# Autodesk Inventor assembly: DriveSide_6inchWheels
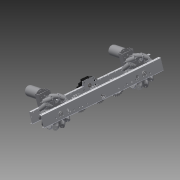
[picture p0: Inventor's stored thumbnail of the model, 180x180]
Saved by Autodesk Inventor 2015 (Build 190159000, 159)
## iProperties
Created: 2016-01-10
Part Number: DriveSide_6inchWheels
Document SubType Name: Assembly
Designer: Applefamily
Author: Applefamily
## Documents named in this file (10)
- C:\Users\Applegate\Desktop\Chassy_Wheeled\Assembly\DriveSide_6inchWheels.iam
- C:\Users\Applegate\Desktop\Chassy_Wheeled\Assembly\Imported Components\am-2951 AM14U2 Outside Sheet.ipt\am-2951 AM14U2 Outside Sheet.ipt.ipt
- C:\Users\Applegate\Desktop\Chassy_Wheeled\Assembly\GearBox and Mec.iam
- C:\Users\Applegate\Desktop\Chassy_Wheeled\Assembly\Imported Components\FR8ZZ Hex Bearing.ipt\FR8ZZ Hex Bearing.ipt.ipt
- C:\Users\Applegate\Desktop\Chassy_Wheeled\Assembly\Imported Components\am-2952 AM14U2 Inside Sheet.ipt\am-2952 AM14U2 Inside Sheet.ipt.ipt
- C:\Users\Applegate\Downloads\Imported Components\4 in HiGrip Wheel\4 in HiGrip Wheel.iam
- C:\Users\Applegate\Downloads\Imported Components\AM14U3+Long+REV1-1\am-2598_107 2016 KOP Toughbox Mini.iam
- am-2951 AM14U2 Outside Sheet.ipt
- FR8ZZ Hex Bearing.ipt
- am-2952 AM14U2 Inside Sheet.ipt
## Components (10 placed, 6 different names)
1. am-2951 AM14U2 Outside Sheet.ipt:1 — Cylindrical:1, Cylindrical:2, Mate:1, Mate:2, Cylindrical:7
2. GearBox and Mec:1 [sub-assembly] — Cylindrical:4, Cylindrical:6, Flush:1, Mate:3
3. FR8ZZ Hex Bearing.ipt:1 — Cylindrical:1, Mate:1, Cylindrical:6
4. FR8ZZ Hex Bearing.ipt:2 — Cylindrical:2, Mate:2, Cylindrical:3
5. GearBox and Mec:2 [sub-assembly] — Cylindrical:3, Cylindrical:5, Flush:1, Mate:4
6. am-2952 AM14U2 Inside Sheet.ipt:1 — Cylindrical:4, Cylindrical:5, Mate:3, Mate:4, Rotational:1
7. 4 in HiGrip Wheel:1 [sub-assembly] — Cylindrical:7, Flush:2, Flush:3
8. 4 in HiGrip Wheel:2 [sub-assembly] — Flush:2
9. 4 in HiGrip Wheel:3 [sub-assembly] — Flush:3
10. am-2598_107 2016 KOP Toughbox Mini:1 [sub-assembly] — Rotational:1
## Relationships (15: CylindricalJoint 7, Mate 4, Flush 3, RevoluteJoint 1)
- Cylindrical:1: am-2951 AM14U2 Outside Sheet.ipt:1 ↔ FR8ZZ Hex Bearing.ipt:1
- Cylindrical:2: am-2951 AM14U2 Outside Sheet.ipt:1 ↔ FR8ZZ Hex Bearing.ipt:2
- Mate:1: am-2951 AM14U2 Outside Sheet.ipt:1 ↔ FR8ZZ Hex Bearing.ipt:1
- Mate:2: am-2951 AM14U2 Outside Sheet.ipt:1 ↔ FR8ZZ Hex Bearing.ipt:2
- Cylindrical:3: FR8ZZ Hex Bearing.ipt:2 ↔ GearBox and Mec:2
- Cylindrical:4: GearBox and Mec:1 ↔ am-2952 AM14U2 Inside Sheet.ipt:1
- Cylindrical:5: GearBox and Mec:2 ↔ am-2952 AM14U2 Inside Sheet.ipt:1
- Cylindrical:6: GearBox and Mec:1 ↔ FR8ZZ Hex Bearing.ipt:1
- Flush:1: GearBox and Mec:1 ↔ GearBox and Mec:2
- Mate:3: GearBox and Mec:1 ↔ am-2952 AM14U2 Inside Sheet.ipt:1
- Mate:4: GearBox and Mec:2 ↔ am-2952 AM14U2 Inside Sheet.ipt:1
- Cylindrical:7: am-2951 AM14U2 Outside Sheet.ipt:1 ↔ 4 in HiGrip Wheel:1
- Flush:2: 4 in HiGrip Wheel:1 ↔ 4 in HiGrip Wheel:2
- Flush:3: 4 in HiGrip Wheel:1 ↔ 4 in HiGrip Wheel:3
- Rotational:1 [RevoluteJoint]: am-2952 AM14U2 Inside Sheet.ipt:1 ↔ am-2598_107 2016 KOP Toughbox Mini:1
